# Autodesk Inventor assembly: Baugruppe1
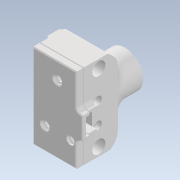
[picture p0: Inventor's stored thumbnail of the model, 180x180]
Saved by Autodesk Inventor 2022.1 (Build 261234020, 234B)
## iProperties
Created: 2022-07-13
Part Number: Baugruppe1
Document SubType Name: Assembly
Designer: Rama
Author: Rama
## Documents named in this file (4)
- C:\Users\Rama\Desktop\GitHub\Voron-2-Mods\Mandalaroseworks\Z_Endstop\CAD\SRC\z_Endstop.iam
- C:\Users\Rama\Desktop\GitHub\Voron-2-Mods\Mandalaroseworks\Z_Endstop\CAD\SRC\housing.ipt
- C:\Users\Rama\Desktop\GitHub\Voron-2-Mods\Mandalaroseworks\Z_Endstop\CAD\SRC\Microswitch_Big.ipt
- C:\Users\Rama\Desktop\GitHub\Voron-2-Mods\Mandalaroseworks\Z_Endstop\CAD\SRC\Buttom_Lid.ipt
## Components (3 placed, 3 different names)
1. housing:1 — Passend:1, Passend:2, Fluchtend:1
2. Microswitch_Big:1 — Passend:1, Passend:2, Winkel:1
3. Buttom_Lid:1 — Fluchtend:1
## Relationships (4: Mate 2, Angle 1, Flush 1)
- Passend:1 [Mate]: housing:1 ↔ Microswitch_Big:1
- Passend:2 [Mate]: housing:1 ↔ Microswitch_Big:1
- Winkel:1 [Angle] (0 deg): Microswitch_Big:1
- Fluchtend:1 [Flush]: housing:1 ↔ Buttom_Lid:1
